# Autodesk Inventor assembly: BearingHousing
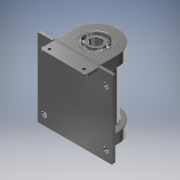
[picture p0: Inventor's stored thumbnail of the model, 180x180]
Saved by Autodesk Inventor 2018 (Build 220112000, 112)
## iProperties
Created: 2018-02-06
Part Number: BearingHousing
Document SubType Name: Weldment
Designer: P136265
Weld Material: Steel, Galvanized
Author: P136265
## Documents named in this file (6)
- C:\Users\P136265\Documents\GitHub\mecanum-cad\BearingHousing.iam
- C:\Users\P136265\Documents\GitHub\mecanum-cad\BearingHousing_Base.ipt
- C:\Users\P136265\Documents\GitHub\mecanum-cad\BearingHousing_Plate.ipt
- C:\Users\P136265\Documents\GitHub\mecanum-cad\BearingHousing_Pipe.ipt
- C:\Users\P136265\Documents\Inventor\Content Center Files\R2018\en-US\SKF B - angular contact\SKF B7204 BE.ipt
- C:\Users\P136265\Documents\GitHub\mecanum-cad\BearingHousing_Jack.ipt
## Components (7 placed, 5 different names)
1. BearingHousing_Base:1 — Mate:2, Mate:3, Mate:4, Mate:5, Mate:6, Mate:7, Mate:14, Mate:15, Mate:16
2. BearingHousing_Plate:1 — Mate:2, Mate:3, Mate:4, Mate:8, Mate:9, Mate:12, Mate:13
3. BearingHousing_Plate:2 — Mate:5, Mate:6, Mate:7, Mate:10, Mate:11
4. BearingHousing_Pipe:1 — Mate:8, Mate:9
5. SKF B- Angular contact SKF B7204 BE:1 — Mate:12, Mate:13
6. SKF B- Angular contact SKF B7204 BE:2 — Mate:10, Mate:11
7. BearingHousing_Jack:1 — Mate:14, Mate:15, Mate:16
## Relationships (15: Mate 15)
- Mate:2 (1 mm): BearingHousing_Base:1 ↔ BearingHousing_Plate:1
- Mate:3: BearingHousing_Base:1 ↔ BearingHousing_Plate:1
- Mate:4: BearingHousing_Base:1 ↔ BearingHousing_Plate:1
- Mate:5: BearingHousing_Base:1 ↔ BearingHousing_Plate:2
- Mate:6 (1 mm): BearingHousing_Base:1 ↔ BearingHousing_Plate:2
- Mate:7: BearingHousing_Base:1 ↔ BearingHousing_Plate:2
- Mate:8: BearingHousing_Plate:1 ↔ BearingHousing_Pipe:1
- Mate:9: BearingHousing_Plate:1 ↔ BearingHousing_Pipe:1
- Mate:10: BearingHousing_Plate:2 ↔ SKF B- Angular contact SKF B7204 BE:2
- Mate:11: BearingHousing_Plate:2 ↔ SKF B- Angular contact SKF B7204 BE:2
- Mate:12: BearingHousing_Plate:1 ↔ SKF B- Angular contact SKF B7204 BE:1
- Mate:13: BearingHousing_Plate:1 ↔ SKF B- Angular contact SKF B7204 BE:1
- Mate:14: BearingHousing_Base:1 ↔ BearingHousing_Jack:1
- Mate:15: BearingHousing_Base:1 ↔ BearingHousing_Jack:1
- Mate:16 (1 mm): BearingHousing_Base:1 ↔ BearingHousing_Jack:1
